# Autodesk Inventor assembly: BBM Staging Plate Assembly
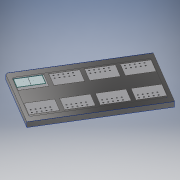
[picture p0: Inventor's stored thumbnail of the model, 180x180]
Saved by Autodesk Inventor 2019.4 (Build 234330000, 330)
## iProperties
Created: 2021-01-11
Part Number: BBM Staging Plate Assembly
Document SubType Name: Assembly
Designer: caleb
Author: caleb
## Documents named in this file (5)
- C:\Users\cfang\Desktop\nebraska-silicon-lab\Hardware\ETL\Module Assembly\BBM Staging Plate\BBM Staging Plate Assembly.iam
- C:\Users\cfang\Desktop\nebraska-silicon-lab\Hardware\ETL\Module Assembly\BBM Staging Plate\BBM Staging Plate.ipt
- C:\Users\cfang\Desktop\nebraska-silicon-lab\Hardware\ETL\Module Assembly\BBM Staging Plate\BBM Staging Plate Stencil.ipt
- C:\Users\cfang\Desktop\nebraska-silicon-lab\Hardware\ETL\Module Assembly\BBM Staging Plate\Bare Bump-Bonded Module.iam
- C:\Users\cfang\Desktop\nebraska-silicon-lab\Hardware\ETL\Module Assembly\BBM Staging Plate\Plastic Inlay.ipt
## Components (4 placed, 4 different names)
1. BBM Staging Plate:1 — Mate:1, Mate:3, Mate:4, Mate:5
2. BBM Staging Plate Stencil:1 — Mate:4
3. Bare Bump-Bonded Module:4 [sub-assembly] — Mate:6
4. Plastic Inlay:1 — Mate:1, Mate:3, Mate:5, Mate:6
## Relationships (5: Mate 5)
- Mate:1: BBM Staging Plate:1 ↔ Plastic Inlay:1
- Mate:3: BBM Staging Plate:1 ↔ Plastic Inlay:1
- Mate:4: BBM Staging Plate:1 ↔ BBM Staging Plate Stencil:1
- Mate:5: BBM Staging Plate:1 ↔ Plastic Inlay:1
- Mate:6: Bare Bump-Bonded Module:4 ↔ Plastic Inlay:1
